# Autodesk Inventor assembly: Carrello semplice
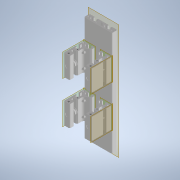
[picture p0: Inventor's stored thumbnail of the model, 180x180]
Saved by Autodesk Inventor 2022 (Build 260153000, 153)
## iProperties
Created: 2021-12-30
Part Number: Carrello semplice
Document SubType Name: Assembly
Designer: matte
Author: matte
## Documents named in this file (3)
- C:\Users\matte\Documents\GitHub\MDM-CyberOrto-CAD\Pezzi singoli\Supporto lineare\Carrello semplice.iam
- C:\Users\matte\Documents\GitHub\MDM-CyberOrto-CAD\Pezzi singoli\Supporto lineare\Piastra-supporto.ipt
- C:\Users\matte\Documents\GitHub\MDM-CyberOrto-CAD\Parker components\08-Linear Application\06-Linear Roller System\01-Roller System 6\30-401.ipt
## Components (5 placed, 2 different names)
1. Piastra-supporto:1
2. 30-401:1
3. 30-401:2
4. 30-401:3
5. 30-401:4
## Relationships (11: Flush 6, Mate 5)
- [Mate]: Piastra-supporto:1 ↔ 30-401:1
- [Flush]: Piastra-supporto:1 ↔ 30-401:1
- [Flush]: Piastra-supporto:1 ↔ 30-401:2
- [Mate]: Piastra-supporto:1 ↔ 30-401:2
- [Mate] (60 mm): 30-401:1 ↔ 30-401:2
- [Mate]: Piastra-supporto:1 ↔ 30-401:3
- [Flush]: Piastra-supporto:1 ↔ 30-401:3
- [Flush]: 30-401:1 ↔ 30-401:3
- [Mate]: Piastra-supporto:1 ↔ 30-401:4
- [Flush]: Piastra-supporto:1 ↔ 30-401:4
- [Flush]: 30-401:2 ↔ 30-401:4
